# Autodesk Inventor assembly: Theremin
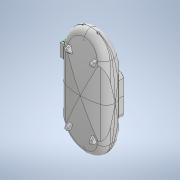
[picture p0: Inventor's stored thumbnail of the model, 180x180]
Saved by Autodesk Inventor 2021 (Build 250183000, 183)
## iProperties
Created: 2020-07-13
Part Number: Theremin
Document SubType Name: Assembly
Designer: chris
Author: chris
## Documents named in this file (9)
- C:\Users\chris\Documents\Christian\3D-Druck\Theremin\Theremin.iam
- C:\Users\chris\Documents\Christian\3D-Druck\Theremin\Theremin_Boden_links.ipt
- C:\Users\chris\Documents\Christian\3D-Druck\Theremin\Theremin_Boden_rechts.ipt
- C:\Users\chris\Documents\Christian\3D-Druck\Theremin\PCB_case.iam
- C:\Users\chris\Documents\Christian\3D-Druck\Theremin\PCB_Theremin.iam
- C:\Users\chris\Documents\Christian\3D-Druck\Theremin\Dummy.ipt
- C:\Users\chris\Documents\Christian\3D-Druck\Theremin\Theremin_Deckel_links.ipt
- C:\Users\chris\Documents\Christian\3D-Druck\Theremin\Theremin_Deckel_rechts.ipt
- C:\Users\chris\Documents\Christian\3D-Druck\Theremin\Stützelement.ipt
## Components (8 placed, 8 different names)
1. Theremin_Boden_links:1 — Passend:1, Passend:2, Passend:3, Passend:4, Passend:5, Passend:6, Passend:7, Passend:8, Passend:9, Passend:10, Passend:11, Passend:12, Passend:13, Passend:14, Fluchtend:1, Passend:15
2. Theremin_Boden_rechts:1 — Passend:1, Passend:2, Passend:3, Passend:16, Passend:18
3. PCB_case:1 [sub-assembly] — Passend:4, Passend:5, Passend:6
4. PCB_Theremin:1 [sub-assembly] — Passend:7, Passend:8, Passend:9, Passend:10
5. Dummy:1 — Passend:11, Passend:12, Passend:13
6. Theremin_Deckel_links:1 — Passend:14, Fluchtend:1, Passend:15, Passend:17, Passend:19, Passend:20, Fluchtend:2
7. Theremin_Deckel_rechts:1 — Passend:16, Passend:17, Passend:18
8. Stützelement:1 — Passend:19, Passend:20, Fluchtend:2
## Relationships (22: Mate 20, Flush 2)
- Passend:1 [Mate] (0.5 mm): Theremin_Boden_links:1 ↔ Theremin_Boden_rechts:1
- Passend:2 [Mate] (0.5 mm): Theremin_Boden_links:1 ↔ Theremin_Boden_rechts:1
- Passend:3 [Mate]: Theremin_Boden_links:1 ↔ Theremin_Boden_rechts:1
- Passend:4 [Mate] (5 mm): Theremin_Boden_links:1 ↔ PCB_case:1
- Passend:5 [Mate] (5 mm): Theremin_Boden_links:1 ↔ PCB_case:1
- Passend:6 [Mate] (1 mm): Theremin_Boden_links:1 ↔ PCB_case:1
- Passend:7 [Mate] (5 mm): Theremin_Boden_links:1 ↔ PCB_Theremin:1
- Passend:8 [Mate] (-5 mm): Theremin_Boden_links:1 ↔ PCB_Theremin:1
- Passend:9 [Mate] (-5 mm): Theremin_Boden_links:1 ↔ PCB_Theremin:1
- Passend:10 [Mate] (-5 mm): Theremin_Boden_links:1 ↔ PCB_Theremin:1
- Passend:11 [Mate] (5 mm): Theremin_Boden_links:1 ↔ Dummy:1
- Passend:12 [Mate]: Theremin_Boden_links:1 ↔ Dummy:1
- Passend:13 [Mate]: Theremin_Boden_links:1 ↔ Dummy:1
- Passend:14 [Mate]: Theremin_Boden_links:1 ↔ Theremin_Deckel_links:1
- Fluchtend:1 [Flush]: Theremin_Boden_links:1 ↔ Theremin_Deckel_links:1
- Passend:15 [Mate]: Theremin_Boden_links:1 ↔ Theremin_Deckel_links:1
- Passend:16 [Mate]: Theremin_Boden_rechts:1 ↔ Theremin_Deckel_rechts:1
- Passend:17 [Mate]: Theremin_Deckel_links:1 ↔ Theremin_Deckel_rechts:1
- Passend:18 [Mate]: Theremin_Boden_rechts:1 ↔ Theremin_Deckel_rechts:1
- Passend:19 [Mate]: Theremin_Deckel_links:1 ↔ Stützelement:1
- Passend:20 [Mate]: Theremin_Deckel_links:1 ↔ Stützelement:1
- Fluchtend:2 [Flush]: Theremin_Deckel_links:1 ↔ Stützelement:1
